# Autodesk Inventor assembly: Assembly of Cover+Plate+Event Camera
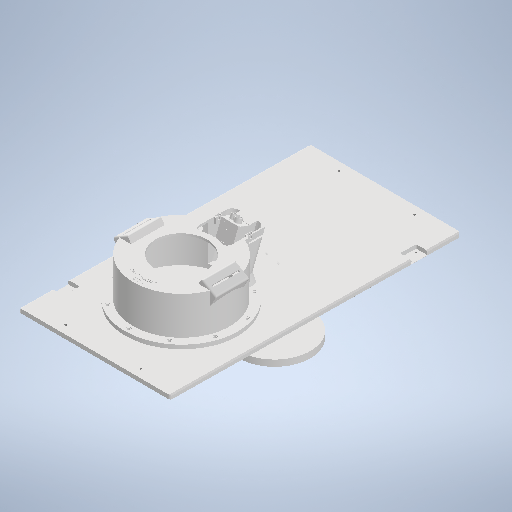
[picture p0: Inventor's stored thumbnail of the model, 512x512]
Saved by Autodesk Inventor 2025 (Build 290162000, 162)
## iProperties
Created: 2026-01-19
Part Number: Assembly of Cover+Plate+Event Camera
Document SubType Name: Assembly
Designer: AdminForWorker
Title: Assembly of Cover+Plate+Event Camera v6
Author: AdminForWorker
## Documents named in this file (7)
- C:\Users\ig2\Desktop\Inventor stuff\Assembly of Cover+Plate+Event Camera.iam
- C:\Users\ig2\Desktop\Inventor stuff\Build Plate v1.ipt
- C:\Users\ig2\Desktop\Inventor stuff\Triton2_Imported v1.ipt
- C:\Users\ig2\Desktop\Inventor stuff\Event Housing v3.ipt
- C:\Users\ig2\Desktop\Inventor stuff\M3 35 mm 18-8 Stainless Steel Socket Head Screw\M3 35 mm 18-8 Stainless Steel Socket Head Screw.ipt
- C:\Users\ig2\Desktop\Inventor stuff\M3 316 Stainless Steel Hex Nut\M3 316 Stainless Steel Hex Nut.ipt
- C:\Users\ig2\Desktop\Inventor stuff\12mm Uru Cover.ipt
## Components (12 placed, 6 different names)
1. Triton2_Imported v1:1 — Rotational:20, Rotational:21, Rotational:22, Rotational:27
2. M3 35 mm 18-8 Stainless Steel Socket Head Screw:1 — Rotational:23
3. M3 35 mm 18-8 Stainless Steel Socket Head Screw:2 — Rotational:24
4. M3 35 mm 18-8 Stainless Steel Socket Head Screw:3 — Rotational:25
5. M3 35 mm 18-8 Stainless Steel Socket Head Screw:4 — Rotational:26
6. M3 316 Stainless Steel Hex Nut:1
7. M3 316 Stainless Steel Hex Nut:2 — Rotational:20
8. M3 316 Stainless Steel Hex Nut:3
9. M3 316 Stainless Steel Hex Nut:4 — Rotational:21
10. 12mm Uru Cover:1 — Mate:1
11. Build Plate v1:1
12. Event Housing v3:1 — Mate:1, Rotational:22, Rotational:23, Rotational:24, Rotational:25, Rotational:26, Rotational:27
## Relationships (9: RevoluteJoint 8, Mate 1)
- Rotational:20 [RevoluteJoint]: Triton2_Imported v1:1 ↔ M3 316 Stainless Steel Hex Nut:2
- Rotational:21 [RevoluteJoint]: Triton2_Imported v1:1 ↔ M3 316 Stainless Steel Hex Nut:4
- Mate:1: 12mm Uru Cover:1 ↔ Event Housing v3:1
- Rotational:22 [RevoluteJoint]: Triton2_Imported v1:1 ↔ Event Housing v3:1
- Rotational:23 [RevoluteJoint]: M3 35 mm 18-8 Stainless Steel Socket Head Screw:1 ↔ Event Housing v3:1
- Rotational:24 [RevoluteJoint]: M3 35 mm 18-8 Stainless Steel Socket Head Screw:2 ↔ Event Housing v3:1
- Rotational:25 [RevoluteJoint]: M3 35 mm 18-8 Stainless Steel Socket Head Screw:3 ↔ Event Housing v3:1
- Rotational:26 [RevoluteJoint]: M3 35 mm 18-8 Stainless Steel Socket Head Screw:4 ↔ Event Housing v3:1
- Rotational:27 [RevoluteJoint]: Triton2_Imported v1:1 ↔ Event Housing v3:1
